# Autodesk Inventor assembly: full
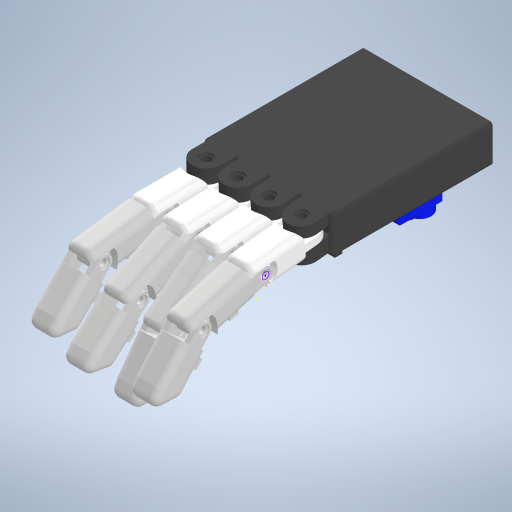
[picture p0: Inventor's stored thumbnail of the model, 512x512]
Saved by Autodesk Inventor 2024 (Build 280153000, 153)
## iProperties
Created: 2023-12-07
Part Number: full
Document SubType Name: Assembly
Designer: stefa
Author: stefa
## Documents named in this file (6)
- S:\ruki\full.iam
- S:\ruki\baze.ipt
- S:\ruki\falanga_big.ipt
- S:\ruki\Servo_SG90.ipt
- S:\ruki\falanga_min.ipt
- S:\ruki\falanga_sm.ipt
## Components (14 placed, 5 different names)
1. baze:1 — Совмещение:1, Совмещение:2, Совмещение:3, Совмещение:4, Совмещение:5, Вставка:1, Вставка:2, Совмещение:18, Совмещение:19, Совмещение:20
2. falanga_big:1 — Совмещение:1, Совмещение:2, Совмещение:3, Совмещение:9
3. falanga_big:2 — Вставка:1, Совмещение:10
4. falanga_big:3 — Вставка:2, Совмещение:11
5. falanga_big:4 — Совмещение:4, Совмещение:5, Совмещение:12
6. Servo_SG90:3 — Совмещение:18, Совмещение:19, Совмещение:20
7. falanga_min:1 — Совмещение:9, Совмещение:16, Совмещение:17
8. falanga_min:2 — Совмещение:10, Совмещение:15
9. falanga_min:3 — Совмещение:12, Совмещение:13
10. falanga_min:4 — Совмещение:11, Совмещение:14
11. falanga_sm:1 — Совмещение:13
12. falanga_sm:2 — Совмещение:15
13. falanga_sm:3 — Совмещение:14
14. falanga_sm:4 — Совмещение:16, Совмещение:17
## Relationships (19: Mate 17, Insert 2)
- Совмещение:1 [Mate]: baze:1 ↔ falanga_big:1
- Совмещение:2 [Mate]: baze:1 ↔ falanga_big:1
- Совмещение:3 [Mate] (5 mm): baze:1 ↔ falanga_big:1
- Совмещение:4 [Mate]: baze:1 ↔ falanga_big:4
- Совмещение:5 [Mate]: baze:1 ↔ falanga_big:4
- Вставка:1 [Insert]: baze:1 ↔ falanga_big:2
- Вставка:2 [Insert]: baze:1 ↔ falanga_big:3
- Совмещение:9 [Mate]: falanga_big:1 ↔ falanga_min:1
- Совмещение:10 [Mate]: falanga_big:2 ↔ falanga_min:2
- Совмещение:11 [Mate]: falanga_big:3 ↔ falanga_min:4
- Совмещение:12 [Mate]: falanga_big:4 ↔ falanga_min:3
- Совмещение:13 [Mate]: falanga_min:3 ↔ falanga_sm:1
- Совмещение:14 [Mate]: falanga_min:4 ↔ falanga_sm:3
- Совмещение:15 [Mate]: falanga_min:2 ↔ falanga_sm:2
- Совмещение:16 [Mate]: falanga_min:1 ↔ falanga_sm:4
- Совмещение:17 [Mate]: falanga_min:1 ↔ falanga_sm:4
- Совмещение:18 [Mate]: baze:1 ↔ Servo_SG90:3
- Совмещение:19 [Mate]: baze:1 ↔ Servo_SG90:3
- Совмещение:20 [Mate]: baze:1 ↔ Servo_SG90:3
